# Autodesk Inventor assembly: 3A.04.05.JS.65.5mm
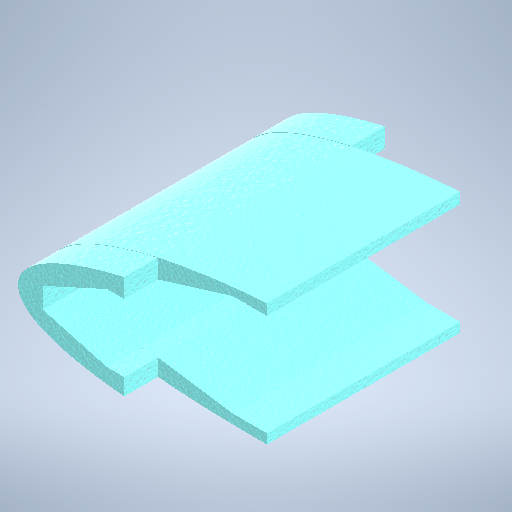
[picture p0: Inventor's stored thumbnail of the model, 512x512]
Saved by Autodesk Inventor 2025.1 (Build 291241000, 241)
## iProperties
Created: 2025-01-14
Part Number: 3A.04.05.JS.65.5mm
Document SubType Name: Assembly
Designer: johan
Author: johan
## Documents named in this file (3)
- C:\Users\johan\OneDrive - University of Bristol\CAD docs\2) Wing\3) Leading edge\assemblies\3A.04.05.JS.65.5mm.iam
- C:\Users\johan\OneDrive - University of Bristol\CAD docs\2) Wing\3) Leading edge\parts\3P.04.JS.2414 rib leading edge v2.ipt
- C:\Users\johan\OneDrive - University of Bristol\CAD docs\2) Wing\3) Leading edge\parts\3P.04.05.JS. leading edge 65.5mm.ipt
## Components (3 placed, 2 different names)
1. 3P.04.JS.2414 rib leading edge v2:1 — Rigid:2
2. 3P.04.JS.2414 rib leading edge v2:2 — Rigid:1
3. 3P.04.05.JS. leading edge 65.5mm:1 — Rigid:1, Rigid:2
## Relationships (2: WeldJoint 2)
- Rigid:1 [WeldJoint]: 3P.04.JS.2414 rib leading edge v2:2 ↔ 3P.04.05.JS. leading edge 65.5mm:1
- Rigid:2 [WeldJoint]: 3P.04.JS.2414 rib leading edge v2:1 ↔ 3P.04.05.JS. leading edge 65.5mm:1
